# Autodesk Inventor assembly: SinnloseKiste
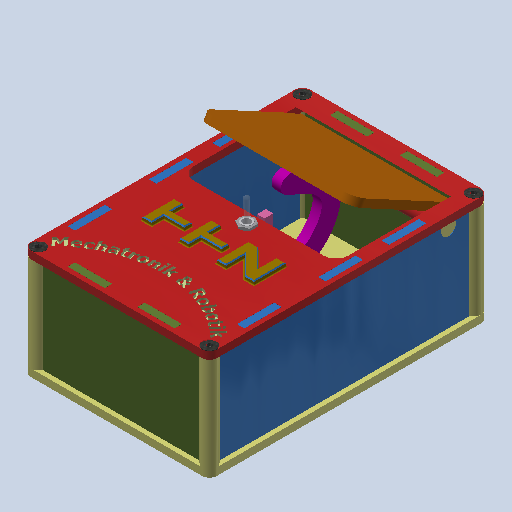
[picture p0: Inventor's stored thumbnail of the model, 512x512]
Saved by Autodesk Inventor 2025.1 (Build 291241000, 241)
## iProperties
Created: 2022-10-31
Part Number: SinnloseKiste
Material: Generisch
Description: STEP AP214
Document SubType Name: Assembly
Designer: RP
Sending System: SolidWorks 2021
Preprocessor: SwSTEP 2.0
Title: _Assembly UM_.STEP
Revision Number: ANY
## Documents named in this file (12)
- C:\Users\Erik\Erik\Hochschule\3. Semester\CAD\CAD-Paspa\Useless Box\_Useless_Box\Useless_Box.iam
- C:\Users\Erik\Erik\Hochschule\3. Semester\CAD\CAD-Paspa\Useless Box\_Useless_Box\SHort panel UM_D‚faut.ipt
- C:\Users\Erik\Erik\Hochschule\3. Semester\CAD\CAD-Paspa\Useless Box\_Useless_Box\Deckplatte.ipt
- C:\Users\Erik\Erik\Hochschule\3. Semester\CAD\CAD-Paspa\Useless Box\_Useless_Box\Klappe.ipt
- C:\Users\Erik\Erik\Hochschule\3. Semester\CAD\CAD-Paspa\Useless Box\_Useless_Box\Seitenteil_lang.ipt
- C:\Users\Erik\Erik\Hochschule\3. Semester\CAD\CAD-Paspa\Useless Box\_Useless_Box\Seitenteil_kurz.ipt
- C:\Users\Erik\Erik\Hochschule\3. Semester\CAD\CAD-Paspa\Useless Box\_Useless_Box\ISO 10642  - M4  x  12.ipt
- C:\Users\Erik\Erik\Hochschule\3. Semester\CAD\CAD-Paspa\Useless Box\_Useless_Box\ISO 10642  - M4  x  16.ipt
- C:\Users\Erik\Erik\Hochschule\3. Semester\CAD\CAD-Paspa\Useless Box\_Useless_Box\Mutter M6x0_5.ipt
- C:\Users\Erik\Erik\Hochschule\3. Semester\CAD\CAD-Paspa\Useless Box\_Useless_Box\Sicherungsscheibe M6.ipt
- C:\Users\Erik\Erik\Hochschule\3. Semester\CAD\CAD-Paspa\Useless Box\_Useless_Box\Antriebseinheit_ZSB.iam
- C:\Users\Erik\Erik\Hochschule\3. Semester\CAD\CAD-Paspa\Useless Box\_Useless_Box\Grundplatte_ZSB.iam
## Components (19 placed, 10 different names)
1. Grundplatte_ZSB:1 [sub-assembly] — Flush:4, Flush:5, Flush:6, Insert:30
2. Antriebseinheit_ZSB:1 [sub-assembly]
3. DIN EN ISO 10642 M4  x  12:1 — Insert:30
4. DIN EN ISO 10642 M4  x  12:2
5. DIN EN ISO 10642 M4  x  12:3
6. DIN EN ISO 10642 M4  x  12:4
7. Mutter M6x0_5:3 — Insert:29
8. Sicherungsscheibe M6 — Insert:29
9. Seitenteil_lang:1
10. Seitenteil_lang:2 — Mate:34
11. Seitenteil_kurz:1
12. Seitenteil_kurz:2
13. Klappe:1 — Mate:34, Mate:39
14. Deckplatte:1 — Mate:39, Insert:17, Insert:18, Insert:19, Insert:20, Insert:27
15. DIN EN ISO 10642 M4  x  16:5 — Insert:17
16. DIN EN ISO 10642 M4  x  16:6 — Insert:20
17. DIN EN ISO 10642 M4  x  16:7 — Insert:18
18. DIN EN ISO 10642 M4  x  16:8 — Insert:19
19. Mutter M6x0_5:2 — Insert:27
## Relationships (38: Mate 20, Insert 12, Flush 4, Angle 1, Tangent 1)
- [Mate]: Grundplatte_ZSB:1 ↔ Seitenteil_lang:1
- [Mate]: Grundplatte_ZSB:1 ↔ Seitenteil_lang:1
- [Mate]: Grundplatte_ZSB:1 ↔ Seitenteil_lang:1
- [Mate]: Grundplatte_ZSB:1 ↔ Seitenteil_lang:2
- [Mate]: Grundplatte_ZSB:1 ↔ Seitenteil_lang:2
- [Mate]: Grundplatte_ZSB:1 ↔ Seitenteil_lang:2
- [Mate]: Grundplatte_ZSB:1 ↔ Seitenteil_kurz:2
- [Mate]: Grundplatte_ZSB:1 ↔ Seitenteil_kurz:2
- [Mate]: Grundplatte_ZSB:1 ↔ Seitenteil_kurz:1
- [Mate]: Grundplatte_ZSB:1 ↔ Seitenteil_kurz:2
- [Mate]: Grundplatte_ZSB:1 ↔ Seitenteil_kurz:1
- [Mate]: Grundplatte_ZSB:1 ↔ Seitenteil_kurz:1
- [Mate]: Grundplatte_ZSB:1 ↔ Seitenteil_kurz:2
- Mate:34: Seitenteil_lang:2 ↔ Klappe:1
- [Insert]: Grundplatte_ZSB:1 ↔ Deckplatte:1
- [Mate]: Grundplatte_ZSB:1 ↔ Deckplatte:1
- [Mate]: Antriebseinheit_ZSB:1 ↔ Deckplatte:1
- [Mate]: Grundplatte_ZSB:1 ↔ Antriebseinheit_ZSB:1
- [Angle] (0 deg): Antriebseinheit_ZSB:1
- [Tangent]: Antriebseinheit_ZSB:1 ↔ Klappe:1
- [Mate]: Antriebseinheit_ZSB:1 ↔ Klappe:1
- Mate:39 (0.1 mm): Klappe:1 ↔ Deckplatte:1
- [Insert]: Grundplatte_ZSB:1 ↔ DIN EN ISO 10642 M4  x  12:2
- [Flush]: Grundplatte_ZSB:1 ↔ DIN EN ISO 10642 M4  x  12:1
- [Insert]: Grundplatte_ZSB:1 ↔ DIN EN ISO 10642 M4  x  12:3
- [Insert]: Grundplatte_ZSB:1 ↔ DIN EN ISO 10642 M4  x  12:4
- Insert:17: Deckplatte:1 ↔ DIN EN ISO 10642 M4  x  16:5
- Insert:18: Deckplatte:1 ↔ DIN EN ISO 10642 M4  x  16:7
- Insert:19: Deckplatte:1 ↔ DIN EN ISO 10642 M4  x  16:8
- Insert:20: Deckplatte:1 ↔ DIN EN ISO 10642 M4  x  16:6
- [Mate]: Antriebseinheit_ZSB:1 ↔ Klappe:1
- Insert:27: Deckplatte:1 ↔ Mutter M6x0_5:2
- [Insert] (0.45 mm): Antriebseinheit_ZSB:1 ↔ Mutter M6x0_5:3
- Insert:29: Mutter M6x0_5:3 ↔ Sicherungsscheibe M6
- Flush:4: Grundplatte_ZSB:1
- Flush:5: Grundplatte_ZSB:1
- Flush:6: Grundplatte_ZSB:1
- Insert:30: Grundplatte_ZSB:1 ↔ DIN EN ISO 10642 M4  x  12:1
